# Autodesk Inventor assembly: Remote Assembly
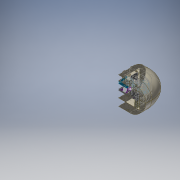
[picture p0: Inventor's stored thumbnail of the model, 180x180]
Saved by Autodesk Inventor 2018 (Build 220112000, 112)
## iProperties
Created: 2015-06-16
Part Number: Remote Assembly
Document SubType Name: Assembly
Designer: Samuel Clay
Author: Samuel Clay
## Documents named in this file (8)
- Z:\enclosure\inventor\Remote Assembly.iam
- Z:\enclosure\inventor\Remote Top.ipt
- Z:\enclosure\inventor\Remote Bottom.ipt
- Z:\enclosure\inventor\Remote Buttons.ipt
- Z:\enclosure\inventor\Case Bottom.ipt
- Z:\enclosure\inventor\Case Top.ipt
- Z:\enclosure\inventor\Case Buttons.ipt
- Z:\enclosure\inventor\Eagle PCB rev 38.ipt
## Components (7 placed, 7 different names)
1. Remote Top:1 — Mate:9, Flush:1, Flush:2, Mate:11, Mate:14
2. Remote Buttons:1 — Mate:6, Insert:1, Mate:14
3. Remote Bottom:1 — Flush:1, Flush:2, Mate:11, Planar:1, Mate:13
4. Case Top:1 — Mate:5, Mate:6, Mate:12
5. Case Bottom:1 — Mate:5, Mate:9, Mate:12, Mate:13
6. Case Buttons:1 — Insert:1
7. Eagle PCB rev 38:1 — Planar:1
## Relationships (11: Mate 7, Flush 2, Insert 1, PlanarJoint 1)
- Mate:5: Case Top:1 ↔ Case Bottom:1
- Mate:6: Remote Buttons:1 ↔ Case Top:1
- Mate:9: Remote Top:1 ↔ Case Bottom:1
- Flush:1: Remote Top:1 ↔ Remote Bottom:1
- Flush:2: Remote Top:1 ↔ Remote Bottom:1
- Mate:11: Remote Top:1 ↔ Remote Bottom:1
- Insert:1: Remote Buttons:1 ↔ Case Buttons:1
- Planar:1: Remote Bottom:1 ↔ Eagle PCB rev 38:1
- Mate:12: Case Top:1 ↔ Case Bottom:1
- Mate:13: Remote Bottom:1 ↔ Case Bottom:1
- Mate:14: Remote Top:1 ↔ Remote Buttons:1
